# Autodesk Inventor assembly: EngineAssembly
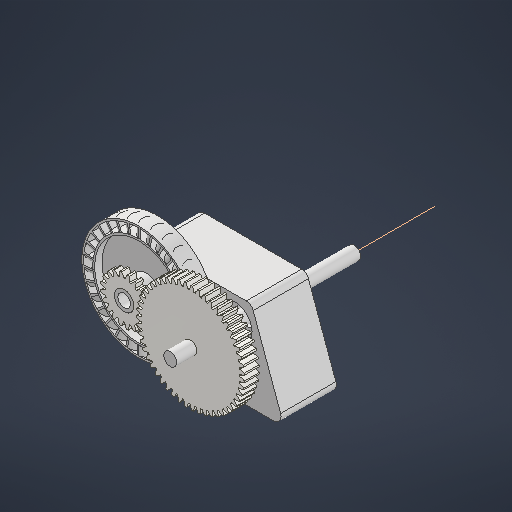
[picture p0: Inventor's stored thumbnail of the model, 512x512]
Saved by Autodesk Inventor 2025.3 (Build 293356030, 356C)
## iProperties
Created: 2025-10-14
Part Number: EngineAssembly
Document SubType Name: Assembly
Designer: yo
Author: yo
## Documents named in this file (5)
- C:\Users\yo\Documents\Andes\9no Semestre\Proyecto Intermedio\Proyecto\Huron-Hudson\Pelton Engine\V7\EngineAssembly.iam
- C:\Users\yo\Documents\Andes\9no Semestre\Proyecto Intermedio\Proyecto\Huron-Hudson\Pelton Engine\V7\Turbine-V3.ipt
- C:\Users\yo\Documents\Andes\9no Semestre\Proyecto Intermedio\Proyecto\Huron-Hudson\Pelton Engine\V7\EngineMount.ipt
- C:\Users\yo\Documents\Andes\9no Semestre\Proyecto Intermedio\Proyecto\Huron-Hudson\Pelton Engine\V7\Shaft.ipt
- C:\Users\yo\Documents\Andes\9no Semestre\Proyecto Intermedio\Proyecto\Huron-Hudson\Pelton Engine\V7\EngineAssembly\Design Accelerator\Spur Gears1.iam
## Components (4 placed, 4 different names)
1. Turbine-V3:1 — Mate:4, Mate:6, Rotation:1, Mate:11, Mate:12, Mate:14
2. EngineMount:1 — Mate:1, Flush:1, Mate:2, Mate:3, Mate:6, Mate:8
3. Shaft:1 — Mate:7, Mate:10, Rotation:2, Mate:13
4. Spur Gears:1 [sub-assembly] — Rotation:1, Rotation:2, Mate:11, Mate:12, Mate:13, Mate:14
## Relationships (17: Mate 14, RelateRotation 2, Flush 1)
- Mate:1: EngineMount:1
- Flush:1: EngineMount:1
- Mate:2: EngineMount:1
- Mate:3: EngineMount:1
- Mate:4: Turbine-V3:1
- Mate:5
- Mate:6: Turbine-V3:1 ↔ EngineMount:1
- Mate:7: Shaft:1
- Mate:8: EngineMount:1
- Mate:9
- Mate:10: Shaft:1
- Rotation:1 [RelateRotation] (1 ul): Turbine-V3:1 ↔ Spur Gears:1
- Rotation:2 [RelateRotation] (1 ul): Shaft:1 ↔ Spur Gears:1
- Mate:11: Turbine-V3:1 ↔ Spur Gears:1
- Mate:12: Turbine-V3:1 ↔ Spur Gears:1
- Mate:13: Shaft:1 ↔ Spur Gears:1
- Mate:14: Turbine-V3:1 ↔ Spur Gears:1
